# Autodesk Inventor assembly: kaiseki2
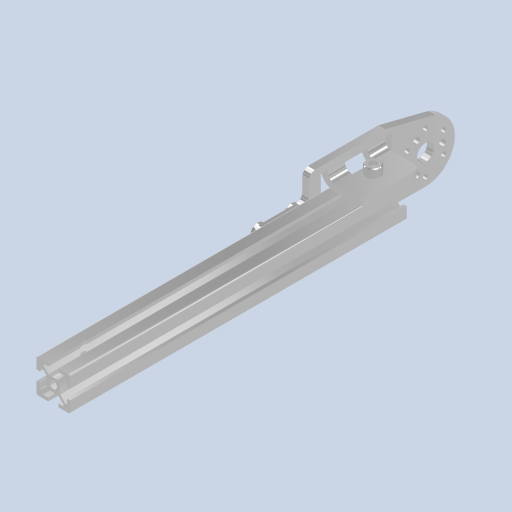
[picture p0: Inventor's stored thumbnail of the model, 512x512]
Saved by Autodesk Inventor 2023 (Build 270158000, 158)
## iProperties
Created: 2024-12-03
Part Number: kaiseki2
Document SubType Name: Assembly
Designer: kiyo
Author: kiyo
## Documents named in this file (12)
- D:\GitHub\inventor\syu-si\OfficeRobot\ReadyMade\Aluminum-frame\test\kaiseki2.iam
- D:\GitHub\inventor\syu-si\OfficeRobot\ReadyMade\Screw\HNTU5-5.ipt
- D:\GitHub\inventor\syu-si\OfficeRobot\ReadyMade\Aluminum-frame\NFS5-2020-200-AV10-BV179.ipt
- D:\GitHub\inventor\syu-si\OfficeRobot\Manipulator\pitch_plate.ipt
- D:\GitHub\inventor\syu-si\OfficeRobot\ReadyMade\Screw\SCB5-25.ipt
- D:\GitHub\inventor\syu-si\OfficeRobot\ReadyMade\Screw\SCB5-10.ipt
- D:\GitHub\inventor\syu-si\OfficeRobot\ReadyMade\Aluminum-frame\test\kaiseki2\AIP\FEA\ewj3gkh28.fins
- D:\GitHub\inventor\syu-si\OfficeRobot\ReadyMade\Aluminum-frame\test\kaiseki2\AIP\FEA\ewj3gkh28.fsat
- D:\GitHub\inventor\syu-si\OfficeRobot\ReadyMade\Aluminum-frame\test\kaiseki2\AIP\FEA\ewj3gkh28.ftes
- D:\GitHub\inventor\syu-si\OfficeRobot\ReadyMade\Aluminum-frame\test\kaiseki2\AIP\FEA\ewj3gkh28.fwiz
- D:\GitHub\inventor\syu-si\OfficeRobot\ReadyMade\Aluminum-frame\test\kaiseki2\AIP\FEA\ewj3gkh40.fmsh
- D:\GitHub\inventor\syu-si\OfficeRobot\ReadyMade\Aluminum-frame\test\kaiseki2\AIP\FEA\ewj3gkh41.fres
## Components (8 placed, 5 different names)
1. HNTU5-5:1 — メイト:16
2. SCB5-10:2 — 正接:7
3. HNTU5-5:2 — メイト:12, 角度:3, メイト:13
4. SCB5-25:1 — メイト:14, 正接:8, 正接:9
5. NFS5-2020-200-AV10-BV179:1 — メイト:9, 角度:2, メイト:11, メイト:12, 角度:3, メイト:13, メイト:15, メイト:16, 角度:4, 角度:5, メイト:17, 正接:8
6. HNTU5-5:3 — メイト:9, 角度:2, メイト:15
7. SCB5-10:1 — 正接:6
8. pitch_plate:1 — メイト:11, メイト:14, 正接:6, 正接:7, メイト:17, 正接:9
## Relationships (21: Mate 10, Tangent 5, Angle 4, Insert 2)
- [Insert] (5.2 mm): HNTU5-5:1 ↔ SCB5-10:2
- [Mate] (1 mm): HNTU5-5:1 ↔ NFS5-2020-200-AV10-BV179:1
- [Mate] (1 mm): HNTU5-5:2 ↔ NFS5-2020-200-AV10-BV179:1
- [Tangent] (7.5 mm): SCB5-25:1 ↔ NFS5-2020-200-AV10-BV179:1
- [Insert] (5.2 mm): HNTU5-5:3 ↔ SCB5-10:1
- メイト:9 [Mate] (1 mm): NFS5-2020-200-AV10-BV179:1 ↔ HNTU5-5:3
- 角度:2 [Angle] (0 deg): NFS5-2020-200-AV10-BV179:1 ↔ HNTU5-5:3
- メイト:11 [Mate]: NFS5-2020-200-AV10-BV179:1 ↔ pitch_plate:1
- メイト:12 [Mate]: HNTU5-5:2 ↔ NFS5-2020-200-AV10-BV179:1
- 角度:3 [Angle] (0 deg): HNTU5-5:2 ↔ NFS5-2020-200-AV10-BV179:1
- メイト:13 [Mate] (1 mm): HNTU5-5:2 ↔ NFS5-2020-200-AV10-BV179:1
- メイト:14 [Mate]: SCB5-25:1 ↔ pitch_plate:1
- メイト:15 [Mate]: NFS5-2020-200-AV10-BV179:1 ↔ HNTU5-5:3
- メイト:16 [Mate]: HNTU5-5:1 ↔ NFS5-2020-200-AV10-BV179:1
- 正接:6 [Tangent] (0.25 mm): SCB5-10:1 ↔ pitch_plate:1
- 正接:7 [Tangent] (0.25 mm): SCB5-10:2 ↔ pitch_plate:1
- 角度:4 [Angle] (0 deg): NFS5-2020-200-AV10-BV179:1
- 角度:5 [Angle] (180 deg): NFS5-2020-200-AV10-BV179:1
- メイト:17 [Mate]: NFS5-2020-200-AV10-BV179:1 ↔ pitch_plate:1
- 正接:8 [Tangent] (7.5 mm): SCB5-25:1 ↔ NFS5-2020-200-AV10-BV179:1
- 正接:9 [Tangent] (0.25 mm): SCB5-25:1 ↔ pitch_plate:1
## Named parameters: d733_d492_d466 = 5.2 mm, d14_d733_d492_d466 = 5.2 mm, sa_0 = 1270, sa_1 = 1270
note: some values were not read from the file. Shown as the stored number, unit unknown: "sa_0", "sa_1".
